# Autodesk Inventor assembly: Tile Field
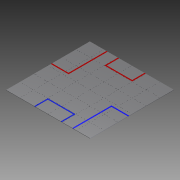
[picture p0: Inventor's stored thumbnail of the model, 180x180]
Saved by Autodesk Inventor 2015 SP1 (Build 190203100, 203)
## iProperties
Category: Field
Company: Autodesk Inc.
Created: 2014-12-18
Document SubType Name: Assembly
Designer: Autodesk Inc.
Catalog Web Link: http://www.usfirst.org/roboticsprograms/ftc/game
Vendor: FIRST
Author: Autodesk Inc.
## Documents named in this file (8)
- D:\Data Folder\FTC 2015\Field Model\Parts\Tile Field.iam
- D:\Data Folder\FTC 2015\Field Model\Parts\Corner soft tile.ipt
- D:\Data Folder\FTC 2015\Field Model\Parts\Side soft tile.ipt
- D:\Data Folder\FTC 2015\Field Model\Parts\Standard soft tile.ipt
- D:\Data Folder\FTC 2015\Field Model\Parts\Floor goal tape.ipt
- D:\Data Folder\FTC 2015\Field Model\Parts\protected zone tape.ipt
- D:\Data Folder\FTC 2015\Field Model\Parts\Floor goal tape_Red.ipt
- D:\Data Folder\FTC 2015\Field Model\Parts\protected zone tape-Red.ipt
## Components (40 placed, 40 different names)
1. Corner soft tile_277
2. Corner soft tile_278
3. Corner soft tile_279 — Symmetry:1
4. Corner soft tile_280 — Symmetry:1
5. Side soft tile_281
6. Side soft tile_282
7. Side soft tile_283
8. Side soft tile_284
9. Side soft tile_285
10. Side soft tile_286
11. Side soft tile_287
12. Side soft tile_288
13. Side soft tile_289
14. Side soft tile_290 — Mate:1, Flush:2
15. Side soft tile_291
16. Side soft tile_292
17. Side soft tile_293
18. Side soft tile_294
19. Side soft tile_295
20. Side soft tile_296
21. Standard soft tile_297
22. Standard soft tile_298
23. Standard soft tile_299
24. Standard soft tile_300
25. Standard soft tile_301
26. Standard soft tile_302
27. Standard soft tile_303
28. Standard soft tile_304
29. Standard soft tile_305
30. Standard soft tile_306
31. Standard soft tile_307
32. Standard soft tile_308
33. Standard soft tile_309
34. Standard soft tile_310
35. Standard soft tile_311
36. Standard soft tile_312
37. Floor goal tape_313
38. protected zone tape_315
39. protected zone tape_316
40. Floor goal tape_Red:1 — Flush:1, Mate:1, Flush:2
## Relationships (4: Flush 2, Symmetry 1, Mate 1)
- Symmetry:1: Corner soft tile_279 ↔ Corner soft tile_280
- Flush:1: Floor goal tape_Red:1
- Mate:1: Side soft tile_290 ↔ Floor goal tape_Red:1
- Flush:2: Side soft tile_290 ↔ Floor goal tape_Red:1
